# Autodesk Inventor assembly: CIM motor 12T thin
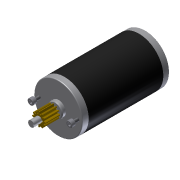
[picture p0: Inventor's stored thumbnail of the model, 180x180]
Saved by Autodesk Inventor 2015 (Build 190159000, 159)
## iProperties
Created: 2011-07-17
Part Number: CIM motor 12T thin
Document SubType Name: Assembly
Designer: Dan Niemitalo
Author: Dan Niemitalo
## Documents named in this file (5)
- H:\Nemo\Documents\Robotics\CAD Files\COTS Parts\Motors\Motor and Pinion Gear Assemblies\CIM motor 12T parametric.iam
- H:\Nemo\Documents\Robotics\CAD Files\COTS Parts\Motors\CIM motor.ipt
- H:\Nemo\Documents\Robotics\CAD Files\COTS Parts\Motors\Motor and Pinion Gear Assemblies\2mmx2mmx10mm_key.ipt
- H:\Nemo\Documents\Robotics\CAD Files\COTS Parts\Gears - VexPro\Gear 20dp 10mm key 12T Vex.ipt
- H:\Nemo\Documents\Robotics\CAD Files\COTS Parts\Fasteners\10-32 SHCS x750.ipt
## Components (5 placed, 4 different names)
1. CIM motor:1 — Mate:3, Mate:4, Mate:5, Angle:1, Insert:1, Insert:2, Mate:6
2. 2mmx2mmx10mm_key:1 — Mate:3, Mate:4
3. Gear 20dp 10mm key 12T Vex:1 — Mate:5, Angle:1, Mate:6
4. 10-32 SHCS x750:1 — Insert:1
5. 10-32 SHCS x750:2 — Insert:2
## Relationships (7: Mate 4, Insert 2, Angle 1)
- Mate:3: CIM motor:1 ↔ 2mmx2mmx10mm_key:1
- Mate:4: CIM motor:1 ↔ 2mmx2mmx10mm_key:1
- Mate:5: CIM motor:1 ↔ Gear 20dp 10mm key 12T Vex:1
- Angle:1 (180 deg): CIM motor:1 ↔ Gear 20dp 10mm key 12T Vex:1
- Insert:1 (6.35 mm): CIM motor:1 ↔ 10-32 SHCS x750:1
- Insert:2 (6.35 mm): CIM motor:1 ↔ 10-32 SHCS x750:2
- Mate:6: CIM motor:1 ↔ Gear 20dp 10mm key 12T Vex:1
